# Autodesk Inventor assembly: mesa_999_001
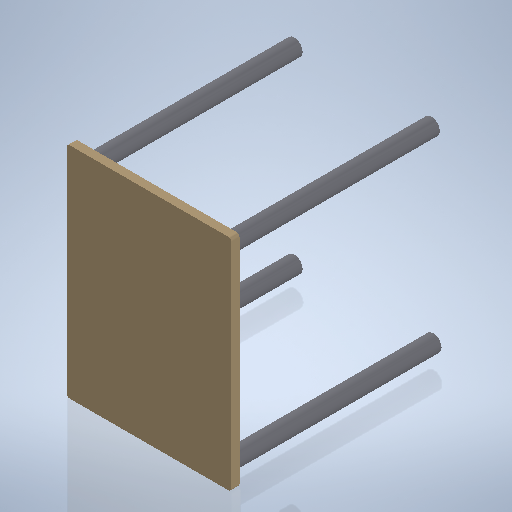
[picture p0: Inventor's stored thumbnail of the model, 512x512]
Saved by Autodesk Inventor 2025.2 (Build 292293000, 293)
## iProperties
Created: 2025-04-02
Part Number: mesa_999_001
Document SubType Name: Assembly
Designer: ishad
Author: ishad
## Documents named in this file (3)
- C:\Users\ishad\Documents\Inventor\Sessao_7\mesa_999_001.iam
- C:\Users\ishad\Documents\Inventor\Sessao_7\Mesa_ergonomica.ipt
- C:\Users\ishad\Documents\Inventor\Sessao_7\peça_001_001.ipt
## Components (5 placed, 2 different names)
1. Mesa_ergonomica:1 — Flush:1, Flush:2, Flush:3, Mate:1
2. peça_001_001:1 — Mate:1, Flush:4, Flush:5, Flush:6, Flush:7, Flush:8, Flush:9, Symmetry:1, Flush:10, Flush:11
3. peça_001_001:2 — Flush:6, Flush:9, Symmetry:1, Flush:12, Flush:13
4. peça_001_001:3 — Flush:7, Flush:12, Flush:13
5. peça_001_001:4 — Flush:8, Flush:10, Flush:11
## Relationships (15: Flush 13, Mate 1, Symmetry 1)
- Flush:1: Mesa_ergonomica:1
- Flush:2: Mesa_ergonomica:1
- Flush:3: Mesa_ergonomica:1
- Mate:1: Mesa_ergonomica:1 ↔ peça_001_001:1
- Flush:4 (250 mm): peça_001_001:1
- Flush:5 (-340 mm): peça_001_001:1
- Flush:6: peça_001_001:1 ↔ peça_001_001:2
- Flush:7: peça_001_001:1 ↔ peça_001_001:3
- Flush:8: peça_001_001:1 ↔ peça_001_001:4
- Flush:9: peça_001_001:1 ↔ peça_001_001:2
- Symmetry:1: peça_001_001:1 ↔ peça_001_001:2
- Flush:10: peça_001_001:1 ↔ peça_001_001:4
- Flush:11 (685.426 mm): peça_001_001:1 ↔ peça_001_001:4
- Flush:12 (-6.573 mm): peça_001_001:2 ↔ peça_001_001:3
- Flush:13 (680.767 mm): peça_001_001:2 ↔ peça_001_001:3
